# Autodesk Inventor assembly: 8133356 CMMT-AS-C7-11A-P3-EP-S1
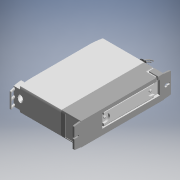
[picture p0: Inventor's stored thumbnail of the model, 180x180]
Saved by Autodesk Inventor 2017.3 (Build 213256000, 256)
## iProperties
Category: PARTsolutions
Company: FESTO
Part Number: 8133356 CMMT-AS-C7-11A-P3-EP-S1
Catalog Web Link: www.cadenas.de
Description: CMMT-servo drive
Vendor: FESTO
Document SubType Name: Assembly
Designer: partserver
Manufacturer: FESTO
Mass: 4100 g
Surface Area: 2500.62 cm^2
Volume: 4194.74 cm^3
Density: 0.977414 g/cm^3
Title: 8133356 CMMT-AS-C7-11A-P3-EP-S1
Author: Cadenas PARTsolutions
Comments: servo drive
PSOL_IDENT_0: {ATYP=ASSISTANT},{DATA=script=$CADENAS_DATA/23d-libs/festo/webfesto.vbb&M_FAMILY=CMMT&M_GROUP=01&M_P
PSOL_IDENT_1: ARTNO=8133356&IDCODE1=CMMT-AS-C7-11A-P3-EP-S1&IDCODE2=&customer_number_cns=&MATES=1&LOD=HI&LOCKERP=0
PSOL_IDENT_2: &SINGLEPART=1}
NB: 8133356 CMMT-AS-C7-11A-P3-EP-S1
NN: CMMT
NT: servo drive
NBSYN: $TNR. $TYP.
LINA: 8133356 CMMT-AS-C7-11A-P3-EP-S1
CATALOG: Festo
TNR: 8133356
TYP: CMMT-AS-C7-11A-P3-EP-S1
B1: 75
B2: 44
B3: 37.5
D1: 11
D2: 5.5
D3: 5.5
H1: 224
H2: 205
L1: 319
L2: 276
L3: 300
L4: 22
L5: 10
L6: 6
L7: 13
CNSMASSEXACT: 4.1
SUPPLIER: FESTO
ARTICLENO: 8133356 CMMT-AS-C7-11A-P3-EP-S1
BOMINFO: 8133356 CMMT-AS-C7-11A-P3-EP-S1
CREATOR: CADENAS GmbH
## Documents named in this file (6)
- e:\temp\worker_7\temp\exporttempdir_6748_144_OBcaO\format_0\8133356 CMMT-AS-C7-11A-P3-EP-S1.iam
- e:\temp\worker_7\temp\exporttempdir_6748_144_OBcaO\format_0\8133356 CMMT-AS-C7-11A-P3-EP-S1---(h).ipt
- e:\temp\worker_7\temp\exporttempdir_6748_144_OBcaO\format_0\5395254 CAFC-C6-C.ipt
- e:\temp\worker_7\temp\exporttempdir_6748_144_OBcaO\format_0\8099429 CMMT-AS-C7_C12-11A-P3---(clamp).ipt
- e:\temp\worker_7\temp\exporttempdir_6748_144_OBcaO\format_0\ISO 14580 M4x25.ipt
- e:\temp\worker_7\temp\exporttempdir_6748_144_OBcaO\format_0\4021832 2GD-1RR7_62-CLP-CBL.ipt
## Components (6 placed, 5 different names)
1. 8133356 CMMT-AS-C7-11A-P3-EP-S1---(h):1 — COVER_XY@1 <-> ANBAU_XY@2, COVER_Z@1 <-> ANBAU_Z@2, COVER_YZ@1 <-> ANBAU_YZ@2, CLAMP_XY@1 <-> ANBAU_XY@3, CLAMP_Z@1 <-> ANBAU_Z@3, CLAMP_YZ@1 <-> ANBAU_YZ@3, PLUG_XY@1 <-> ANBAU_XY@6, PLUG_Z@1 <-> ANBAU_Z@6, PLUG_YZ@1 <-> ANBAU_YZ@6
2. 5395254 CAFC-C6-C:1 — COVER_XY@1 <-> ANBAU_XY@2, COVER_Z@1 <-> ANBAU_Z@2, COVER_YZ@1 <-> ANBAU_YZ@2
3. 8099429 CMMT-AS-C7_C12-11A-P3---(clamp):1 — CLAMP_XY@1 <-> ANBAU_XY@3, CLAMP_Z@1 <-> ANBAU_Z@3, CLAMP_YZ@1 <-> ANBAU_YZ@3, SCREW_1_XY@3 <-> IP1_XY@4, SCREW_1_Z@3 <-> IP1_Z@4, SCREW_1_YZ@3 <-> IP1_YZ@4, SCREW_2_XY@3 <-> IP1_XY@5, SCREW_2_Z@3 <-> IP1_Z@5, SCREW_2_YZ@3 <-> IP1_YZ@5
4. ISO 14580 M4x25:1 — SCREW_1_XY@3 <-> IP1_XY@4, SCREW_1_Z@3 <-> IP1_Z@4, SCREW_1_YZ@3 <-> IP1_YZ@4
5. ISO 14580 M4x25:2 — SCREW_2_XY@3 <-> IP1_XY@5, SCREW_2_Z@3 <-> IP1_Z@5, SCREW_2_YZ@3 <-> IP1_YZ@5
6. 4021832 2GD-1RR7_62-CLP-CBL:1 — PLUG_XY@1 <-> ANBAU_XY@6, PLUG_Z@1 <-> ANBAU_Z@6, PLUG_YZ@1 <-> ANBAU_YZ@6
## Relationships (15: Mate 10, Angle 5)
- COVER_XY@1 <-> ANBAU_XY@2 [Mate]: 8133356 CMMT-AS-C7-11A-P3-EP-S1---(h):1 ↔ 5395254 CAFC-C6-C:1
- COVER_Z@1 <-> ANBAU_Z@2 [Mate]: 8133356 CMMT-AS-C7-11A-P3-EP-S1---(h):1 ↔ 5395254 CAFC-C6-C:1
- COVER_YZ@1 <-> ANBAU_YZ@2 [Angle] (0 deg): 8133356 CMMT-AS-C7-11A-P3-EP-S1---(h):1 ↔ 5395254 CAFC-C6-C:1
- CLAMP_XY@1 <-> ANBAU_XY@3 [Mate]: 8133356 CMMT-AS-C7-11A-P3-EP-S1---(h):1 ↔ 8099429 CMMT-AS-C7_C12-11A-P3---(clamp):1
- CLAMP_Z@1 <-> ANBAU_Z@3 [Mate]: 8133356 CMMT-AS-C7-11A-P3-EP-S1---(h):1 ↔ 8099429 CMMT-AS-C7_C12-11A-P3---(clamp):1
- CLAMP_YZ@1 <-> ANBAU_YZ@3 [Angle] (0 deg): 8133356 CMMT-AS-C7-11A-P3-EP-S1---(h):1 ↔ 8099429 CMMT-AS-C7_C12-11A-P3---(clamp):1
- SCREW_1_XY@3 <-> IP1_XY@4 [Mate]: 8099429 CMMT-AS-C7_C12-11A-P3---(clamp):1 ↔ ISO 14580 M4x25:1
- SCREW_1_Z@3 <-> IP1_Z@4 [Mate]: 8099429 CMMT-AS-C7_C12-11A-P3---(clamp):1 ↔ ISO 14580 M4x25:1
- SCREW_1_YZ@3 <-> IP1_YZ@4 [Angle] (0 deg): 8099429 CMMT-AS-C7_C12-11A-P3---(clamp):1 ↔ ISO 14580 M4x25:1
- SCREW_2_XY@3 <-> IP1_XY@5 [Mate]: 8099429 CMMT-AS-C7_C12-11A-P3---(clamp):1 ↔ ISO 14580 M4x25:2
- SCREW_2_Z@3 <-> IP1_Z@5 [Mate]: 8099429 CMMT-AS-C7_C12-11A-P3---(clamp):1 ↔ ISO 14580 M4x25:2
- SCREW_2_YZ@3 <-> IP1_YZ@5 [Angle] (0 deg): 8099429 CMMT-AS-C7_C12-11A-P3---(clamp):1 ↔ ISO 14580 M4x25:2
- PLUG_XY@1 <-> ANBAU_XY@6 [Mate]: 8133356 CMMT-AS-C7-11A-P3-EP-S1---(h):1 ↔ 4021832 2GD-1RR7_62-CLP-CBL:1
- PLUG_Z@1 <-> ANBAU_Z@6 [Mate]: 8133356 CMMT-AS-C7-11A-P3-EP-S1---(h):1 ↔ 4021832 2GD-1RR7_62-CLP-CBL:1
- PLUG_YZ@1 <-> ANBAU_YZ@6 [Angle] (0 deg): 8133356 CMMT-AS-C7-11A-P3-EP-S1---(h):1 ↔ 4021832 2GD-1RR7_62-CLP-CBL:1
